# Autodesk Inventor assembly: 000 Ensamblaje 3d_JacintoDevKit_Addon - BASIC
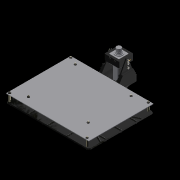
[picture p0: Inventor's stored thumbnail of the model, 180x180]
Saved by Autodesk Inventor 2018.3 (Build 223284000, 284)
## iProperties
Category: 0
Created: 2025-11-24
Part Number: 000 Ensamblaje 3d_JacintoDevKit_Addon - BASIC
Document SubType Name: Assembly
Designer: mbs18
Manufacturer-1: {"Link": "", "Name": "Embention Sistemas Inteligentes S.A.", "PartNumber": "3d_JacintoDevKit_Addon - BASIC", "partner_id": false}
Manufacturer-2: {"Link": "", "Name": "", "PartNumber": "", "partner_id": false}
Manufacturer-3: {"Link": "", "Name": "", "PartNumber": "", "partner_id": false}
Manufacturer-4: {"Link": "", "Name": "", "PartNumber": "", "partner_id": false}
Manufacturer-5: {"Link": "", "Name": "", "PartNumber": "", "partner_id": false}
Provider-1: {"Link": "", "Name": "", "PartNumber": "", "partner_id": false}
Provider-2: {"Link": "", "Name": "", "PartNumber": "", "partner_id": false}
Provider-3: {"Link": "", "Name": "", "PartNumber": "", "partner_id": false}
Provider-4: {"Link": "", "Name": "", "PartNumber": "", "partner_id": false}
Provider-5: {"Link": "", "Name": "", "PartNumber": "", "partner_id": false}
odoo_id: 18673
odoo_item_code: 3d_JacintoDevKit_Addon
odoo_internal_code: P014366
odoo_pt_internal_code: PT11508
odoo_part_number_code: 3d_JacintoDevKit_Addon/BASIC-101010
odoo_model: product.template
odoo_x2o_application_version: 12.0.4.20
odoo_d2o_version: 12.0.1.6.0
Author: mbs18
## Documents named in this file (16)
- C:\Users\aca6\git\DAA\items\JacintoDevKit_Addon\items\3d_JacintoDevKit_Addon\variants\BASIC\3d\000 Ensamblaje 3d_JacintoDevKit_Addon - BASIC.iam
- C:\Users\aca6\git\DAA\items\JacintoDevKit_Addon\items\3d_JacintoDevKit_Addon\3d\3d_JacintoDevKit_Addon - base.ipt
- C:\Users\aca6\git\DAA\items\JacintoDevKit_Addon\items\3d_JacintoDevKit_Addon\3d\3d_JacintoDevKit_Addon - Panel bracket.ipt
- C:\Users\aca6\git\DAA\items\_accessories\Tornilleria\Insertos\3d_PennEngineering_(SI)\3d\PPB-M3-1.ipt
- C:\Users\aca6\git\DAA\items\_accessories\Separadores y torretas\Internal\Brass\3d_Harwin\3d\R30-3001902 (M3x19 male-female).ipt
- C:\Users\aca6\git\DAA\items\_accessories\Tornilleria\Tornillos\3d_DIN 912\3d\A4 Black Inox\DIN 912 - M3 x 0,5 x 8 - Black INOX.ipt
- C:\Users\aca6\git\DAA\items\_accessories\Separadores y torretas\Internal\Steel\3d_Wurth\3d\970200471 (M4x20).ipt
- C:\Users\aca6\git\DAA\items\_accessories\Tornilleria\Tornillos\3d_DIN 912\3d\A4 Black Inox\DIN 912 - M4 x 0,7 x 10 - Black INOX.ipt
- C:\Users\aca6\git\DAA\items\_accessories\Tornilleria\Tornillos\3d_DIN 7991\3d\A4 Black Inox\DIN 7991 - M3x8 Black INOX.ipt
- C:\Users\aca6\git\DAA\items\_accessories\Tornilleria\Arandelas\3d_DIN 125 A\3d\A4 Black INOX\DIN 125 - A 3,2 Black INOX.ipt
- C:\Users\aca6\git\DAA\items\_accessories\Tornilleria\Arandelas\3d_DIN 125 A\3d\A4 Black INOX\DIN 125 - A 4,3 Black INOX.ipt
- C:\Users\aca6\git\DAA\items\_accessories\Tornilleria\Arandelas\3d_DIN 127\3d\A4 Black Inox\DIN 127 - A3 Black INOX.ipt
- C:\Users\aca6\git\DAA\items\JacintoDevKit_Addon\items\3d_JacintoDevKit_Addon\3d\3d_JacintoDevKit_Addon - Camera.ipt
- C:\Users\aca6\git\DAA\items\JacintoDevKit_Addon\items\3d_JacintoDevKit_Addon\3d\3d_JacintoDevKit_Addon - USB Type-C.ipt
- C:\Users\aca6\git\DAA\items\JacintoDevKit_Addon\items\3d_JacintoDevKit_Addon\3d\3d_JacintoDevKit_Addon - Jacinto.ipt
- C:\Users\aca6\git\DAA\items\_accessories\Tornilleria\Tornillos\3d_DIN 912\3d\A4 Inox\DIN 912 - M3 x 0,5 x 8 -  INOX.ipt
## Components (79 placed, 15 different names)
1. 3d_JacintoDevKit_Addon - Camera:1 — Flush:32, Mate:196, Mate:197, Mate:204, Mate:205, Mate:206
2. 3d_JacintoDevKit_Addon - USB Type-C:1 — Mate:204, Mate:205, Mate:206
3. 3d_JacintoDevKit_Addon - Jacinto:1 — Mate:212, Flush:33, Flush:34
4. 3d_JacintoDevKit_Addon - base:1 — Mate:1, Mate:2, Flush:1, Mate:67, Mate:75, Mate:76, Mate:77, Mate:78, Mate:79, Mate:80, Mate:81, Mate:82, Mate:83, Mate:84, Mate:85, Mate:86, Mate:87, Mate:88, Mate:89, Mate:90, Mate:91, Mate:92, Mate:93, Mate:94, Mate:95, Mate:96, Mate:97, Mate:98, Mate:99, Mate:100, Mate:101, Mate:102, Mate:104, Mate:105, Mate:106, Mate:156, Mate:160, Mate:161, Mate:162, Mate:179, Mate:181, Mate:183, Mate:185, Mate:187, Mate:189, Mate:191, Mate:193, Mate:207, Mate:208, Mate:209, Mate:210, Mate:211, Mate:212, Flush:33, Flush:34, Angle:1, Mate:217, Mate:218, Mate:219, Mate:222, Mate:224, Mate:227, Mate:228, Mate:229, Mate:230, Mate:233, Mate:234, Mate:235, Mate:236, Mate:237, Mate:239
5. 3d_JacintoDevKit_Addon - Panel bracket:1 — Flush:8, Flush:9, Flush:32, Mate:196, Mate:197, Mate:198, Tangent:1, Mate:199, Tangent:2, Mate:200, Tangent:3, Mate:201, Tangent:4, Mate:202, Mate:203, Mate:209, Mate:213, Mate:214, Flush:35, Flush:36, Angle:1, Mate:215, Flush:37, Flush:38, Mate:226
6. PPB-M3-1:3 — Mate:213, Flush:35
7. PPB-M3-1:4 — Mate:214, Flush:36
8. PPB-M3-1:5 — Mate:215, Flush:38
9. PPB-M3-1:6 — Flush:37, Mate:221, Mate:226
10. DIN 912 - M3 x 0,5 x 8 -  INOX:1 — Mate:219, Mate:220
11. DIN 912 - M3 x 0,5 x 8 -  INOX:2 — Mate:221, Mate:222, Mate:223, Mate:225
12. DIN 127 - A3 Black INOX:3 — Mate:223, Mate:224, Mate:225
13. DIN 127 - A3 Black INOX:4 — Mate:227, Mate:228, Mate:232
14. DIN 912 - M3 x 0,5 x 8 -  INOX:3 — Mate:230, Mate:231
15. DIN 912 - M3 x 0,5 x 8 -  INOX:4 — Mate:229, Mate:232
16. DIN 912 - M3 x 0,5 x 8 -  INOX:5 — Mate:237, Mate:238
17. DIN 912 - M3 x 0,5 x 8 -  INOX:6 — Mate:239, Mate:240
18. DIN 127 - A3 Black INOX:5 — Mate:233, Mate:234, Mate:240
19. DIN 127 - A3 Black INOX:6 — Mate:235, Mate:236, Mate:238
20. DIN 125 - A 3,2 Black INOX:17 — Mate:180, Mate:181
21. DIN 125 - A 3,2 Black INOX:18 — Mate:182, Mate:183
22. DIN 125 - A 3,2 Black INOX:19 — Mate:184, Mate:185
23. DIN 125 - A 3,2 Black INOX:20 — Mate:178, Mate:179
24. DIN 125 - A 3,2 Black INOX:21 — Mate:188, Mate:189
25. DIN 125 - A 3,2 Black INOX:22 — Mate:192, Mate:193
26. DIN 125 - A 3,2 Black INOX:23 — Mate:190, Mate:191
27. DIN 125 - A 3,2 Black INOX:24 — Mate:186, Mate:187
28. PPB-M3-1:1 — Flush:8, Mate:202, Mate:207, Mate:208
29. PPB-M3-1:2 — Flush:9, Mate:203
30. DIN 7991 - M3x8 Black INOX:1 — Mate:198, Tangent:1
31. DIN 7991 - M3x8 Black INOX:2 — Mate:201, Tangent:4
32. DIN 7991 - M3x8 Black INOX:3 — Mate:199, Tangent:2
33. DIN 7991 - M3x8 Black INOX:4 — Mate:200, Tangent:3
34. R30-3001902 (M3x19 male-female):1 — Mate:67, Mate:75, Flush:17, Flush:18, Flush:19, Mate:147, Mate:149
35. R30-3001902 (M3x19 male-female):2 — Mate:77, Flush:18, Flush:20, Mate:129, Mate:130
36. R30-3001902 (M3x19 male-female):3 — Mate:76, Flush:17, Mate:148, Mate:150
37. R30-3001902 (M3x19 male-female):4 — Mate:78, Flush:19, Mate:123, Mate:124, Mate:125
38. R30-3001902 (M3x19 male-female):5 — Mate:79, Flush:20, Flush:21, Mate:151, Mate:152
39. R30-3001902 (M3x19 male-female):6 — Mate:83, Flush:22, Mate:137, Mate:138
40. R30-3001902 (M3x19 male-female):7 — Mate:81, Mate:82, Flush:22, Mate:135, Mate:136
41. R30-3001902 (M3x19 male-female):8 — Mate:80, Flush:21, Mate:153, Mate:154
42. DIN 912 - M3 x 0,5 x 8 - Black INOX:1 — Mate:84, Mate:85, Flush:23, Mate:178
43. DIN 912 - M3 x 0,5 x 8 - Black INOX:2 — Flush:24, Mate:88, Mate:190
44. DIN 912 - M3 x 0,5 x 8 - Black INOX:3 — Mate:86, Flush:23, Flush:25, Flush:28, Mate:180
45. DIN 912 - M3 x 0,5 x 8 - Black INOX:4 — Flush:24, Mate:87, Flush:25, Mate:192
46. DIN 912 - M3 x 0,5 x 8 - Black INOX:5 — Mate:89, Flush:26, Flush:27, Flush:28, Mate:182
47. DIN 912 - M3 x 0,5 x 8 - Black INOX:6 — Mate:91, Flush:26, Mate:188
48. DIN 912 - M3 x 0,5 x 8 - Black INOX:7 — Mate:90, Flush:27, Mate:184
49. DIN 912 - M3 x 0,5 x 8 - Black INOX:8 — Mate:92, Mate:93, Mate:186
50. 970200471 (M4x20):1 — Mate:94, Mate:95
51. 970200471 (M4x20):2 — Mate:100, Mate:101
52. 970200471 (M4x20):3 — Mate:98, Mate:99
53. 970200471 (M4x20):4 — Mate:96, Mate:97
54. DIN 912 - M4 x 0,7 x 10 - Black INOX:1 — Mate:102, Mate:103, Flush:29, Mate:155
55. DIN 912 - M4 x 0,7 x 10 - Black INOX:2 — Mate:106, Flush:29, Flush:30, Mate:158
56. DIN 912 - M4 x 0,7 x 10 - Black INOX:3 — Mate:105, Flush:30, Flush:31, Mate:159
57. DIN 912 - M4 x 0,7 x 10 - Black INOX:4 — Mate:104, Flush:31, Mate:157
58. DIN 125 - A 3,2 Black INOX:1 — Mate:124, Mate:125, Mate:126
59. DIN 125 - A 3,2 Black INOX:2 — Mate:123, Mate:126
60. DIN 125 - A 3,2 Black INOX:3 — Mate:128, Mate:129, Mate:130
61. DIN 125 - A 3,2 Black INOX:4 — Mate:128
62. DIN 125 - A 3,2 Black INOX:5 — Mate:135, Mate:136
63. DIN 125 - A 3,2 Black INOX:6
64. DIN 125 - A 3,2 Black INOX:7 — Mate:138
65. DIN 125 - A 3,2 Black INOX:8 — Mate:137
66. DIN 125 - A 3,2 Black INOX:9 — Mate:153, Mate:154
67. DIN 125 - A 3,2 Black INOX:10
68. DIN 125 - A 3,2 Black INOX:11 — Mate:151, Mate:152
69. DIN 125 - A 3,2 Black INOX:12
70. DIN 125 - A 3,2 Black INOX:13 — Mate:148, Mate:150
71. DIN 125 - A 3,2 Black INOX:14
72. DIN 125 - A 3,2 Black INOX:15 — Mate:147, Mate:149
73. DIN 125 - A 3,2 Black INOX:16
74. DIN 125 - A 4,3 Black INOX:1 — Mate:155, Mate:156, Mate:103
75. DIN 125 - A 4,3 Black INOX:2 — Mate:157, Mate:161
76. DIN 125 - A 4,3 Black INOX:3 — Mate:159, Mate:160
77. DIN 125 - A 4,3 Black INOX:4 — Mate:158, Mate:162
78. DIN 127 - A3 Black INOX:1 — Mate:210, Mate:218, Mate:220
79. DIN 127 - A3 Black INOX:2 — Mate:211, Mate:217, Mate:231
## Relationships (165: Mate 135, Flush 25, Tangent 4, Angle 1)
- Mate:1: 3d_JacintoDevKit_Addon - base:1
- Mate:2: 3d_JacintoDevKit_Addon - base:1
- Flush:1: 3d_JacintoDevKit_Addon - base:1
- Flush:8 (0.2 mm): 3d_JacintoDevKit_Addon - Panel bracket:1 ↔ PPB-M3-1:1
- Flush:9: 3d_JacintoDevKit_Addon - Panel bracket:1 ↔ PPB-M3-1:2
- Mate:67: 3d_JacintoDevKit_Addon - base:1 ↔ R30-3001902 (M3x19 male-female):1
- Mate:75: 3d_JacintoDevKit_Addon - base:1 ↔ R30-3001902 (M3x19 male-female):1
- Mate:76: 3d_JacintoDevKit_Addon - base:1 ↔ R30-3001902 (M3x19 male-female):3
- Flush:17: R30-3001902 (M3x19 male-female):1 ↔ R30-3001902 (M3x19 male-female):3
- Mate:77: 3d_JacintoDevKit_Addon - base:1 ↔ R30-3001902 (M3x19 male-female):2
- Mate:78: 3d_JacintoDevKit_Addon - base:1 ↔ R30-3001902 (M3x19 male-female):4
- Flush:18: R30-3001902 (M3x19 male-female):1 ↔ R30-3001902 (M3x19 male-female):2
- Flush:19: R30-3001902 (M3x19 male-female):1 ↔ R30-3001902 (M3x19 male-female):4
- Mate:79: 3d_JacintoDevKit_Addon - base:1 ↔ R30-3001902 (M3x19 male-female):5
- Flush:20: R30-3001902 (M3x19 male-female):2 ↔ R30-3001902 (M3x19 male-female):5
- Mate:80: 3d_JacintoDevKit_Addon - base:1 ↔ R30-3001902 (M3x19 male-female):8
- Flush:21: R30-3001902 (M3x19 male-female):5 ↔ R30-3001902 (M3x19 male-female):8
- Mate:81: 3d_JacintoDevKit_Addon - base:1 ↔ R30-3001902 (M3x19 male-female):7
- Mate:82: 3d_JacintoDevKit_Addon - base:1 ↔ R30-3001902 (M3x19 male-female):7
- Mate:83: 3d_JacintoDevKit_Addon - base:1 ↔ R30-3001902 (M3x19 male-female):6
- Flush:22: R30-3001902 (M3x19 male-female):6 ↔ R30-3001902 (M3x19 male-female):7
- Mate:84: 3d_JacintoDevKit_Addon - base:1 ↔ DIN 912 - M3 x 0,5 x 8 - Black INOX:1
- Mate:85: 3d_JacintoDevKit_Addon - base:1 ↔ DIN 912 - M3 x 0,5 x 8 - Black INOX:1
- Mate:86: 3d_JacintoDevKit_Addon - base:1 ↔ DIN 912 - M3 x 0,5 x 8 - Black INOX:3
- Flush:23: DIN 912 - M3 x 0,5 x 8 - Black INOX:1 ↔ DIN 912 - M3 x 0,5 x 8 - Black INOX:3
- Flush:24: DIN 912 - M3 x 0,5 x 8 - Black INOX:2 ↔ DIN 912 - M3 x 0,5 x 8 - Black INOX:4
- Mate:87: 3d_JacintoDevKit_Addon - base:1 ↔ DIN 912 - M3 x 0,5 x 8 - Black INOX:4
- Flush:25: DIN 912 - M3 x 0,5 x 8 - Black INOX:3 ↔ DIN 912 - M3 x 0,5 x 8 - Black INOX:4
- Mate:88: 3d_JacintoDevKit_Addon - base:1 ↔ DIN 912 - M3 x 0,5 x 8 - Black INOX:2
- Mate:89: 3d_JacintoDevKit_Addon - base:1 ↔ DIN 912 - M3 x 0,5 x 8 - Black INOX:5
- Mate:90: 3d_JacintoDevKit_Addon - base:1 ↔ DIN 912 - M3 x 0,5 x 8 - Black INOX:7
- Mate:91: 3d_JacintoDevKit_Addon - base:1 ↔ DIN 912 - M3 x 0,5 x 8 - Black INOX:6
- Flush:26: DIN 912 - M3 x 0,5 x 8 - Black INOX:5 ↔ DIN 912 - M3 x 0,5 x 8 - Black INOX:6
- Flush:27: DIN 912 - M3 x 0,5 x 8 - Black INOX:5 ↔ DIN 912 - M3 x 0,5 x 8 - Black INOX:7
- Flush:28: DIN 912 - M3 x 0,5 x 8 - Black INOX:3 ↔ DIN 912 - M3 x 0,5 x 8 - Black INOX:5
- Mate:92: 3d_JacintoDevKit_Addon - base:1 ↔ DIN 912 - M3 x 0,5 x 8 - Black INOX:8
- Mate:93: 3d_JacintoDevKit_Addon - base:1 ↔ DIN 912 - M3 x 0,5 x 8 - Black INOX:8
- Mate:94: 3d_JacintoDevKit_Addon - base:1 ↔ 970200471 (M4x20):1
- Mate:95: 3d_JacintoDevKit_Addon - base:1 ↔ 970200471 (M4x20):1
- Mate:96: 3d_JacintoDevKit_Addon - base:1 ↔ 970200471 (M4x20):4
- Mate:97: 3d_JacintoDevKit_Addon - base:1 ↔ 970200471 (M4x20):4
- Mate:98: 3d_JacintoDevKit_Addon - base:1 ↔ 970200471 (M4x20):3
- Mate:99: 3d_JacintoDevKit_Addon - base:1 ↔ 970200471 (M4x20):3
- Mate:100: 3d_JacintoDevKit_Addon - base:1 ↔ 970200471 (M4x20):2
- Mate:101: 3d_JacintoDevKit_Addon - base:1 ↔ 970200471 (M4x20):2
- Mate:102: 3d_JacintoDevKit_Addon - base:1 ↔ DIN 912 - M4 x 0,7 x 10 - Black INOX:1
- Mate:103: DIN 912 - M4 x 0,7 x 10 - Black INOX:1 ↔ DIN 125 - A 4,3 Black INOX:1
- Mate:104: 3d_JacintoDevKit_Addon - base:1 ↔ DIN 912 - M4 x 0,7 x 10 - Black INOX:4
- Mate:105: 3d_JacintoDevKit_Addon - base:1 ↔ DIN 912 - M4 x 0,7 x 10 - Black INOX:3
- Mate:106: 3d_JacintoDevKit_Addon - base:1 ↔ DIN 912 - M4 x 0,7 x 10 - Black INOX:2
- Flush:29: DIN 912 - M4 x 0,7 x 10 - Black INOX:1 ↔ DIN 912 - M4 x 0,7 x 10 - Black INOX:2
- Flush:30: DIN 912 - M4 x 0,7 x 10 - Black INOX:2 ↔ DIN 912 - M4 x 0,7 x 10 - Black INOX:3
- Flush:31: DIN 912 - M4 x 0,7 x 10 - Black INOX:3 ↔ DIN 912 - M4 x 0,7 x 10 - Black INOX:4
- Mate:123: R30-3001902 (M3x19 male-female):4 ↔ DIN 125 - A 3,2 Black INOX:2
- Mate:124: R30-3001902 (M3x19 male-female):4 ↔ DIN 125 - A 3,2 Black INOX:1
- Mate:125: R30-3001902 (M3x19 male-female):4 ↔ DIN 125 - A 3,2 Black INOX:1
- Mate:126 (1.6 mm): DIN 125 - A 3,2 Black INOX:1 ↔ DIN 125 - A 3,2 Black INOX:2
- [Mate] (1.6 mm): DIN 125 - A 3,2 Black INOX:3 ↔ DIN 125 - A 3,2 Black INOX:4
- Mate:128: DIN 125 - A 3,2 Black INOX:3 ↔ DIN 125 - A 3,2 Black INOX:4
- Mate:129: R30-3001902 (M3x19 male-female):2 ↔ DIN 125 - A 3,2 Black INOX:3
- Mate:130: R30-3001902 (M3x19 male-female):2 ↔ DIN 125 - A 3,2 Black INOX:3
- [Mate] (1.6 mm): DIN 125 - A 3,2 Black INOX:5 ↔ DIN 125 - A 3,2 Black INOX:6
- [Mate]: DIN 125 - A 3,2 Black INOX:5 ↔ DIN 125 - A 3,2 Black INOX:6
- [Mate] (1.6 mm): DIN 125 - A 3,2 Black INOX:7 ↔ DIN 125 - A 3,2 Black INOX:8
- [Mate]: DIN 125 - A 3,2 Black INOX:7 ↔ DIN 125 - A 3,2 Black INOX:8
- Mate:135: R30-3001902 (M3x19 male-female):7 ↔ DIN 125 - A 3,2 Black INOX:5
- Mate:136: R30-3001902 (M3x19 male-female):7 ↔ DIN 125 - A 3,2 Black INOX:5
- Mate:137: R30-3001902 (M3x19 male-female):6 ↔ DIN 125 - A 3,2 Black INOX:8
- Mate:138: R30-3001902 (M3x19 male-female):6 ↔ DIN 125 - A 3,2 Black INOX:7
- [Mate] (1.6 mm): DIN 125 - A 3,2 Black INOX:9 ↔ DIN 125 - A 3,2 Black INOX:10
- [Mate]: DIN 125 - A 3,2 Black INOX:9 ↔ DIN 125 - A 3,2 Black INOX:10
- [Mate] (1.6 mm): DIN 125 - A 3,2 Black INOX:11 ↔ DIN 125 - A 3,2 Black INOX:12
- [Mate]: DIN 125 - A 3,2 Black INOX:11 ↔ DIN 125 - A 3,2 Black INOX:12
- [Mate] (1.6 mm): DIN 125 - A 3,2 Black INOX:13 ↔ DIN 125 - A 3,2 Black INOX:14
- [Mate]: DIN 125 - A 3,2 Black INOX:13 ↔ DIN 125 - A 3,2 Black INOX:14
- [Mate] (1.6 mm): DIN 125 - A 3,2 Black INOX:15 ↔ DIN 125 - A 3,2 Black INOX:16
- [Mate]: DIN 125 - A 3,2 Black INOX:15 ↔ DIN 125 - A 3,2 Black INOX:16
- Mate:147: R30-3001902 (M3x19 male-female):1 ↔ DIN 125 - A 3,2 Black INOX:15
- Mate:148: R30-3001902 (M3x19 male-female):3 ↔ DIN 125 - A 3,2 Black INOX:13
- Mate:149: R30-3001902 (M3x19 male-female):1 ↔ DIN 125 - A 3,2 Black INOX:15
- Mate:150: R30-3001902 (M3x19 male-female):3 ↔ DIN 125 - A 3,2 Black INOX:13
- Mate:151: R30-3001902 (M3x19 male-female):5 ↔ DIN 125 - A 3,2 Black INOX:11
- Mate:152: R30-3001902 (M3x19 male-female):5 ↔ DIN 125 - A 3,2 Black INOX:11
- Mate:153: R30-3001902 (M3x19 male-female):8 ↔ DIN 125 - A 3,2 Black INOX:9
- Mate:154: R30-3001902 (M3x19 male-female):8 ↔ DIN 125 - A 3,2 Black INOX:9
- Mate:155: DIN 912 - M4 x 0,7 x 10 - Black INOX:1 ↔ DIN 125 - A 4,3 Black INOX:1
- Mate:156: 3d_JacintoDevKit_Addon - base:1 ↔ DIN 125 - A 4,3 Black INOX:1
- Mate:157: DIN 912 - M4 x 0,7 x 10 - Black INOX:4 ↔ DIN 125 - A 4,3 Black INOX:2
- Mate:158: DIN 912 - M4 x 0,7 x 10 - Black INOX:2 ↔ DIN 125 - A 4,3 Black INOX:4
- Mate:159: DIN 912 - M4 x 0,7 x 10 - Black INOX:3 ↔ DIN 125 - A 4,3 Black INOX:3
- Mate:160: 3d_JacintoDevKit_Addon - base:1 ↔ DIN 125 - A 4,3 Black INOX:3
- Mate:161: 3d_JacintoDevKit_Addon - base:1 ↔ DIN 125 - A 4,3 Black INOX:2
- Mate:162: 3d_JacintoDevKit_Addon - base:1 ↔ DIN 125 - A 4,3 Black INOX:4
- Mate:178: DIN 125 - A 3,2 Black INOX:20 ↔ DIN 912 - M3 x 0,5 x 8 - Black INOX:1
- Mate:179: 3d_JacintoDevKit_Addon - base:1 ↔ DIN 125 - A 3,2 Black INOX:20
- Mate:180: DIN 125 - A 3,2 Black INOX:17 ↔ DIN 912 - M3 x 0,5 x 8 - Black INOX:3
- Mate:181: 3d_JacintoDevKit_Addon - base:1 ↔ DIN 125 - A 3,2 Black INOX:17
- Mate:182: DIN 125 - A 3,2 Black INOX:18 ↔ DIN 912 - M3 x 0,5 x 8 - Black INOX:5
- Mate:183: 3d_JacintoDevKit_Addon - base:1 ↔ DIN 125 - A 3,2 Black INOX:18
- Mate:184: DIN 125 - A 3,2 Black INOX:19 ↔ DIN 912 - M3 x 0,5 x 8 - Black INOX:7
- Mate:185: 3d_JacintoDevKit_Addon - base:1 ↔ DIN 125 - A 3,2 Black INOX:19
- Mate:186: DIN 125 - A 3,2 Black INOX:24 ↔ DIN 912 - M3 x 0,5 x 8 - Black INOX:8
- Mate:187: 3d_JacintoDevKit_Addon - base:1 ↔ DIN 125 - A 3,2 Black INOX:24
- Mate:188: DIN 125 - A 3,2 Black INOX:21 ↔ DIN 912 - M3 x 0,5 x 8 - Black INOX:6
- Mate:189: 3d_JacintoDevKit_Addon - base:1 ↔ DIN 125 - A 3,2 Black INOX:21
- Mate:190: DIN 125 - A 3,2 Black INOX:23 ↔ DIN 912 - M3 x 0,5 x 8 - Black INOX:2
- Mate:191: 3d_JacintoDevKit_Addon - base:1 ↔ DIN 125 - A 3,2 Black INOX:23
- Mate:192: DIN 125 - A 3,2 Black INOX:22 ↔ DIN 912 - M3 x 0,5 x 8 - Black INOX:4
- Mate:193: 3d_JacintoDevKit_Addon - base:1 ↔ DIN 125 - A 3,2 Black INOX:22
- Flush:32: 3d_JacintoDevKit_Addon - Camera:1 ↔ 3d_JacintoDevKit_Addon - Panel bracket:1
- Mate:196 (0.15 mm): 3d_JacintoDevKit_Addon - Camera:1 ↔ 3d_JacintoDevKit_Addon - Panel bracket:1
- Mate:197 (0.15 mm): 3d_JacintoDevKit_Addon - Camera:1 ↔ 3d_JacintoDevKit_Addon - Panel bracket:1
- Mate:198: 3d_JacintoDevKit_Addon - Panel bracket:1 ↔ DIN 7991 - M3x8 Black INOX:1
- Tangent:1: 3d_JacintoDevKit_Addon - Panel bracket:1 ↔ DIN 7991 - M3x8 Black INOX:1
- Mate:199: 3d_JacintoDevKit_Addon - Panel bracket:1 ↔ DIN 7991 - M3x8 Black INOX:3
- Tangent:2: 3d_JacintoDevKit_Addon - Panel bracket:1 ↔ DIN 7991 - M3x8 Black INOX:3
- Mate:200: 3d_JacintoDevKit_Addon - Panel bracket:1 ↔ DIN 7991 - M3x8 Black INOX:4
- Tangent:3: 3d_JacintoDevKit_Addon - Panel bracket:1 ↔ DIN 7991 - M3x8 Black INOX:4
- Mate:201: 3d_JacintoDevKit_Addon - Panel bracket:1 ↔ DIN 7991 - M3x8 Black INOX:2
- Tangent:4: 3d_JacintoDevKit_Addon - Panel bracket:1 ↔ DIN 7991 - M3x8 Black INOX:2
- Mate:202: 3d_JacintoDevKit_Addon - Panel bracket:1 ↔ PPB-M3-1:1
- Mate:203: 3d_JacintoDevKit_Addon - Panel bracket:1 ↔ PPB-M3-1:2
- Mate:204: 3d_JacintoDevKit_Addon - Camera:1 ↔ 3d_JacintoDevKit_Addon - USB Type-C:1
- Mate:205: 3d_JacintoDevKit_Addon - Camera:1 ↔ 3d_JacintoDevKit_Addon - USB Type-C:1
- Mate:206: 3d_JacintoDevKit_Addon - Camera:1 ↔ 3d_JacintoDevKit_Addon - USB Type-C:1
- Mate:207: 3d_JacintoDevKit_Addon - base:1 ↔ PPB-M3-1:1
- Mate:208: 3d_JacintoDevKit_Addon - base:1 ↔ PPB-M3-1:1
- Mate:209 (0.3 mm): 3d_JacintoDevKit_Addon - base:1 ↔ 3d_JacintoDevKit_Addon - Panel bracket:1
- Mate:210: 3d_JacintoDevKit_Addon - base:1 ↔ DIN 127 - A3 Black INOX:1
- Mate:211: 3d_JacintoDevKit_Addon - base:1 ↔ DIN 127 - A3 Black INOX:2
- Mate:212 (19.5 mm): 3d_JacintoDevKit_Addon - Jacinto:1 ↔ 3d_JacintoDevKit_Addon - base:1
- Flush:33: 3d_JacintoDevKit_Addon - Jacinto:1 ↔ 3d_JacintoDevKit_Addon - base:1
- Flush:34: 3d_JacintoDevKit_Addon - Jacinto:1 ↔ 3d_JacintoDevKit_Addon - base:1
- Mate:213: 3d_JacintoDevKit_Addon - Panel bracket:1 ↔ PPB-M3-1:3
- Mate:214: 3d_JacintoDevKit_Addon - Panel bracket:1 ↔ PPB-M3-1:4
- Flush:35: 3d_JacintoDevKit_Addon - Panel bracket:1 ↔ PPB-M3-1:3
- Flush:36: 3d_JacintoDevKit_Addon - Panel bracket:1 ↔ PPB-M3-1:4
- Angle:1 (0 deg): 3d_JacintoDevKit_Addon - base:1 ↔ 3d_JacintoDevKit_Addon - Panel bracket:1
- Mate:215: 3d_JacintoDevKit_Addon - Panel bracket:1 ↔ PPB-M3-1:5
- Flush:37: 3d_JacintoDevKit_Addon - Panel bracket:1 ↔ PPB-M3-1:6
- Flush:38: 3d_JacintoDevKit_Addon - Panel bracket:1 ↔ PPB-M3-1:5
- Mate:217: 3d_JacintoDevKit_Addon - base:1 ↔ DIN 127 - A3 Black INOX:2
- Mate:218: 3d_JacintoDevKit_Addon - base:1 ↔ DIN 127 - A3 Black INOX:1
- Mate:219: 3d_JacintoDevKit_Addon - base:1 ↔ DIN 912 - M3 x 0,5 x 8 -  INOX:1
- Mate:220: DIN 912 - M3 x 0,5 x 8 -  INOX:1 ↔ DIN 127 - A3 Black INOX:1
- Mate:221: PPB-M3-1:6 ↔ DIN 912 - M3 x 0,5 x 8 -  INOX:2
- Mate:222: 3d_JacintoDevKit_Addon - base:1 ↔ DIN 912 - M3 x 0,5 x 8 -  INOX:2
- Mate:223: DIN 912 - M3 x 0,5 x 8 -  INOX:2 ↔ DIN 127 - A3 Black INOX:3
- Mate:224: 3d_JacintoDevKit_Addon - base:1 ↔ DIN 127 - A3 Black INOX:3
- Mate:225: DIN 912 - M3 x 0,5 x 8 -  INOX:2 ↔ DIN 127 - A3 Black INOX:3
- Mate:226: 3d_JacintoDevKit_Addon - Panel bracket:1 ↔ PPB-M3-1:6
- Mate:227: 3d_JacintoDevKit_Addon - base:1 ↔ DIN 127 - A3 Black INOX:4
- Mate:228: 3d_JacintoDevKit_Addon - base:1 ↔ DIN 127 - A3 Black INOX:4
- Mate:229: 3d_JacintoDevKit_Addon - base:1 ↔ DIN 912 - M3 x 0,5 x 8 -  INOX:4
- Mate:230: 3d_JacintoDevKit_Addon - base:1 ↔ DIN 912 - M3 x 0,5 x 8 -  INOX:3
- Mate:231: DIN 912 - M3 x 0,5 x 8 -  INOX:3 ↔ DIN 127 - A3 Black INOX:2
- Mate:232: DIN 127 - A3 Black INOX:4 ↔ DIN 912 - M3 x 0,5 x 8 -  INOX:4
- Mate:233: 3d_JacintoDevKit_Addon - base:1 ↔ DIN 127 - A3 Black INOX:5
- Mate:234: 3d_JacintoDevKit_Addon - base:1 ↔ DIN 127 - A3 Black INOX:5
- Mate:235: 3d_JacintoDevKit_Addon - base:1 ↔ DIN 127 - A3 Black INOX:6
- Mate:236: 3d_JacintoDevKit_Addon - base:1 ↔ DIN 127 - A3 Black INOX:6
- Mate:237: 3d_JacintoDevKit_Addon - base:1 ↔ DIN 912 - M3 x 0,5 x 8 -  INOX:5
- Mate:238: DIN 912 - M3 x 0,5 x 8 -  INOX:5 ↔ DIN 127 - A3 Black INOX:6
- Mate:239: 3d_JacintoDevKit_Addon - base:1 ↔ DIN 912 - M3 x 0,5 x 8 -  INOX:6
- Mate:240: DIN 912 - M3 x 0,5 x 8 -  INOX:6 ↔ DIN 127 - A3 Black INOX:5
## Named parameters: d174_d173 = 1.6 mm, d178_d174_d173 = 1.6 mm, d179_d175 = 0 mm, d180_d174_d173 = 1.6 mm, d181_d175 = 0 mm, d186_d174_d173 = 1.6 mm, d187_d175 = 0 mm, d188_d174_d173 = 1.6 mm, d189_d175 = 0 mm, d190_d174_d173 = 1.6 mm, d191_d175 = 0 mm, d192_d174_d173 = 1.6 mm, d193_d175 = 0 mm
